# Autodesk Inventor assembly: Wolley Wheel
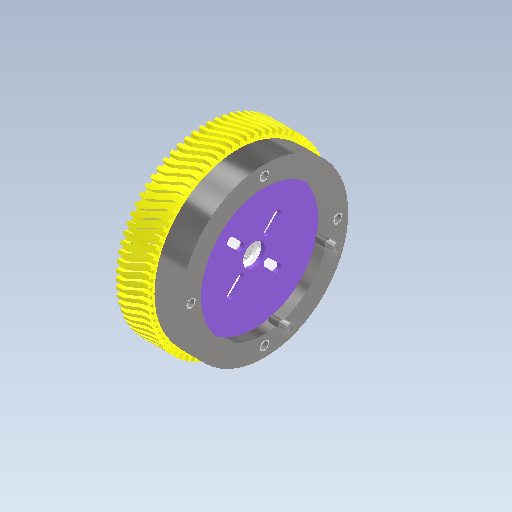
[picture p0: Inventor's stored thumbnail of the model, 512x512]
Saved by Autodesk Inventor 2021 (Build 250183000, 183)
## iProperties
Created: 2021-02-27
Part Number: Wolley Wheel
Document SubType Name: Assembly
Designer: Jack
Author: Jack
Title: Wolley Wheel
## Documents named in this file (37)
- C:\Users\Jack\Projekt\Wolley\MEC_SpeedReducerWheel\SpeedReducerWheel.iam
- C:\Users\Jack\Projekt\Wolley\MEC_SpeedReducerWheel\Back.ipt
- C:\Users\Jack\Projekt\Wolley\MEC_SpeedReducerWheel\RingGearA.ipt
- C:\Users\Jack\Projekt\Wolley\MEC_SpeedReducerWheel\SunGearA.ipt
- C:\Users\Jack\Projekt\Wolley\MEC_SpeedReducerWheel\PlanetGearA.ipt
- C:\Users\Jack\Projekt\Wolley\MEC_SpeedReducerWheel\Middle.ipt
- C:\Users\Jack\Projekt\Wolley\MEC_SpeedReducerWheel\PCB.ipt
- C:\Users\Jack\Projekt\Wolley\MEC_SpeedReducerWheel\Carrier.ipt
- C:\Users\Jack\Projekt\Wolley\MEC_SpeedReducerWheel\Shaft1.ipt
- C:\Users\Jack\Projekt\Wolley\MEC_SpeedReducerWheel\Shaft2.ipt
- C:\Users\Jack\Projekt\Wolley\MEC_SpeedReducerWheel\CarrierB.ipt
- C:\Users\Jack\Projekt\Wolley\MEC_SpeedReducerWheel\Front.ipt
- C:\Users\Jack\Projekt\Wolley\MEC_SpeedReducerWheel\Wheel.ipt
- C:\Users\Jack\Projekt\Wolley\MEC_SpeedReducerWheel\SunGearB.ipt
- C:\Users\Jack\Projekt\Wolley\MEC_SpeedReducerWheel\Tire.ipt
- C:\Users\Jack\Projekt\Wolley\MEC_SpeedReducerWheel\Enclosure.ipt
- C:\Users\Jack\Projekt\Wolley\MEC_SpeedReducerWheel\PlanetGearB.ipt
- C:\Users\Jack\Projekt\Wolley\MEC_SpeedReducerWheel\Mount.ipt
- C:\Users\Jack\Projekt\Wolley\MEC_SpeedReducerWheel\SpeedReducerWheel\Design Accelerator\RingGearA_SpurGears.iam
- C:\Users\Jack\Projekt\Wolley\MEC_SpeedReducerWheel\SpeedReducerWheel\Design Accelerator\PlanetGearA_SpurGears2.iam
- C:\Users\Jack\Projekt\Wolley\MEC_SpeedReducerWheel\SpeedReducerWheel\Design Accelerator\SunGearB_SpurGears1.iam
- C:\Users\Jack\Projekt\Wolley\MEC_SpeedReducerWheel\SpeedReducerWheel\Design Accelerator\PlanetGearB_SpurGears1.iam
- C:\Users\Jack\Projekt\Wolley\MEC_SpeedReducerWheel\SpeedReducerWheel\Design Accelerator\RingGearB_SpurGears.iam
- C:\Users\Jack\Projekt\Wolley\MEC_SpeedReducerWheel\PlanetGearB_CPY.ipt
- C:\Users\Jack\Projekt\Wolley\MEC_SpeedReducerWheel\PlanetGearB_CPY1.ipt
- C:\Users\Jack\Documents\Inventor\Content Center Files\R2021\en-US\DIN 912\DIN 912 - M3 x 0,5 x 5 x 3,75.ipt
- C:\Users\Jack\Projekt\Wolley\MEC_SpeedReducerWheel\MiddleStandoff.ipt
- C:\Users\Jack\Projekt\Wolley\MEC_SpeedReducerWheel\SpeedReducerWheel\Design Accelerator\SunGearA_SpurGears2.iam
- C:\Users\Jack\Projekt\Wolley\MEC_SpeedReducerWheel\Shaft1_1.ipt
- C:\Users\Jack\Projekt\Wolley\MEC_SpeedReducerWheel\Magnet.ipt
- C:\Users\Jack\Projekt\Wolley\MEC_SpeedReducerWheel\Magnet_CPY.ipt
- C:\Users\Jack\Projekt\Wolley\MEC_SpeedReducerWheel\Magnet_CPY1.ipt
- C:\Users\Jack\Documents\Inventor\Content Center Files\R2021\en-US\DIN 912\DIN 912 - M3 x 0,5 x 6 x 4,75.ipt
- C:\Users\Jack\Projekt\Wolley\MEC_SpeedReducerWheel\PlanetGearA_CPY2.ipt
- C:\Users\Jack\Projekt\Wolley\MEC_SpeedReducerWheel\PlanetGearA_CPY3.ipt
- C:\Users\Jack\Documents\Inventor\Content Center Files\R2021\en-US\DIN 912\DIN 912 - M3 x 0,5 x 16 x 14,75.ipt
- C:\Users\Jack\Projekt\Wolley\MEC_SpeedReducerWheel\M3ThreadedInsert.ipt
## Components (54 placed, 36 different names)
1. Back:1
2. RingGearA:1
3. SunGearA:1 — Flush:1, Mate:2
4. PlanetGearA:1 — Rotational:1, Flush:1
5. Middle:1 — Mate:1, Rotational:5, Rotational:6, Insert:1, Insert:2, Insert:3, Rotational:16, Rotational:17, Rotational:18, Insert:4, Insert:5, Insert:6, Insert:7
6. PCB:1
7. Carrier:1 — Rotational:1, Rigid:2, Rigid:3, Rigid:4, Rotational:19, Rotational:20
8. Shaft1:1
9. Shaft2:1
10. CarrierB:1 — Mate:3, Mate:5, Mate:7, Rotational:9, Rotational:10, Rotational:11
11. Front:1 — Mate:4, Mate:6, Mate:8
12. Wheel:1 — Rotational:6, Rigid:1
13. SunGearB:1 — Rotational:5
14. Tire:1 — Rigid:1
15. Enclosure:1 — Rigid:5, Rigid:6, Rigid:7, Rigid:8
16. PlanetGearB:1 — Rotational:9
17. Mount:1
18. RingGearA_SpurGears:1 [sub-assembly]
19. PlanetGearA_SpurGears:1 [sub-assembly]
20. SunGearB_SpurGears:1 [sub-assembly]
21. PlanetGearB_SpurGears:1 [sub-assembly]
22. RingGearB_SpurGears:1 [sub-assembly]
23. PlanetGearB_CPY:1 — Rotational:10
24. PlanetGearB_CPY1:1 — Rotational:11
25. DIN 912 - replaced by DIN EN ISO 4762 M3 x 5:1 — Mate:3, Mate:4
26. DIN 912 - replaced by DIN EN ISO 4762 M3 x 5:2 — Mate:5, Mate:6
27. DIN 912 - replaced by DIN EN ISO 4762 M3 x 5:3 — Mate:7, Mate:8
28. DIN 912 - replaced by DIN EN ISO 4762 M3 x 5:4 — Insert:1
29. DIN 912 - replaced by DIN EN ISO 4762 M3 x 5:5 — Insert:2
30. DIN 912 - replaced by DIN EN ISO 4762 M3 x 5:6 — Insert:3
31. SunGearA_SpurGears2:1 [sub-assembly]
32. Shaft1_1:1
33. Magnet:1 — Rigid:2
34. Magnet_CPY:1 — Rigid:3
35. Magnet_CPY1:1 — Rigid:4
36. DIN 912 - replaced by DIN EN ISO 4762 M3 x 6:3
37. DIN 912 - replaced by DIN EN ISO 4762 M3 x 6:4
38. MiddleStandoff:9 — Rotational:16
39. MiddleStandoff:10 — Rotational:17
40. MiddleStandoff:11 — Rotational:18
41. PlanetGearA_CPY2:1 — Rotational:19
42. PlanetGearA_CPY3:1 — Rotational:20
43. DIN 912 - replaced by DIN EN ISO 4762 M3 x 16:1 — Insert:4
44. DIN 912 - replaced by DIN EN ISO 4762 M3 x 16:2 — Insert:5
45. DIN 912 - replaced by DIN EN ISO 4762 M3 x 16:3 — Insert:6
46. DIN 912 - replaced by DIN EN ISO 4762 M3 x 16:4 — Insert:7
47. M3ThreadedInsert:1 — Rigid:5
48. M3ThreadedInsert:2 — Rigid:6
49. M3ThreadedInsert:3 — Rigid:7
50. M3ThreadedInsert:4 — Rigid:8
51. MiddleStandoff:1
52. MiddleStandoff:2
53. MiddleStandoff:3
54. MiddleStandoff:4
## Component patterns: (4 elements, first: MiddleStandoff:1)
## Relationships (35: RevoluteJoint 11, Mate 8, WeldJoint 8, Insert 7, Flush 1)
- Rotational:1 [RevoluteJoint] (1 mm): PlanetGearA:1 ↔ Carrier:1
- Mate:1: Middle:1
- Flush:1: SunGearA:1 ↔ PlanetGearA:1
- Mate:2: SunGearA:1
- Rotational:5 [RevoluteJoint]: Middle:1 ↔ SunGearB:1
- Rotational:6 [RevoluteJoint]: Middle:1 ↔ Wheel:1
- Rigid:1 [WeldJoint]: Wheel:1 ↔ Tire:1
- Mate:3: CarrierB:1 ↔ DIN 912 - replaced by DIN EN ISO 4762 M3 x 5:1
- Mate:4: Front:1 ↔ DIN 912 - replaced by DIN EN ISO 4762 M3 x 5:1
- Mate:5: CarrierB:1 ↔ DIN 912 - replaced by DIN EN ISO 4762 M3 x 5:2
- Mate:6: Front:1 ↔ DIN 912 - replaced by DIN EN ISO 4762 M3 x 5:2
- Mate:7: CarrierB:1 ↔ DIN 912 - replaced by DIN EN ISO 4762 M3 x 5:3
- Mate:8: Front:1 ↔ DIN 912 - replaced by DIN EN ISO 4762 M3 x 5:3
- Insert:1: Middle:1 ↔ DIN 912 - replaced by DIN EN ISO 4762 M3 x 5:4
- Insert:2: Middle:1 ↔ DIN 912 - replaced by DIN EN ISO 4762 M3 x 5:5
- Insert:3: Middle:1 ↔ DIN 912 - replaced by DIN EN ISO 4762 M3 x 5:6
- Rotational:9 [RevoluteJoint]: CarrierB:1 ↔ PlanetGearB:1
- Rotational:10 [RevoluteJoint]: CarrierB:1 ↔ PlanetGearB_CPY:1
- Rotational:11 [RevoluteJoint]: CarrierB:1 ↔ PlanetGearB_CPY1:1
- Rigid:2 [WeldJoint]: Carrier:1 ↔ Magnet:1
- Rigid:3 [WeldJoint]: Carrier:1 ↔ Magnet_CPY:1
- Rigid:4 [WeldJoint]: Carrier:1 ↔ Magnet_CPY1:1
- Rotational:16 [RevoluteJoint]: Middle:1 ↔ MiddleStandoff:9
- Rotational:17 [RevoluteJoint]: Middle:1 ↔ MiddleStandoff:10
- Rotational:18 [RevoluteJoint]: Middle:1 ↔ MiddleStandoff:11
- Rotational:19 [RevoluteJoint]: Carrier:1 ↔ PlanetGearA_CPY2:1
- Rotational:20 [RevoluteJoint]: Carrier:1 ↔ PlanetGearA_CPY3:1
- Insert:4: Middle:1 ↔ DIN 912 - replaced by DIN EN ISO 4762 M3 x 16:1
- Insert:5: Middle:1 ↔ DIN 912 - replaced by DIN EN ISO 4762 M3 x 16:2
- Insert:6: Middle:1 ↔ DIN 912 - replaced by DIN EN ISO 4762 M3 x 16:3
- Insert:7: Middle:1 ↔ DIN 912 - replaced by DIN EN ISO 4762 M3 x 16:4
- Rigid:5 [WeldJoint]: Enclosure:1 ↔ M3ThreadedInsert:1
- Rigid:6 [WeldJoint]: Enclosure:1 ↔ M3ThreadedInsert:2
- Rigid:7 [WeldJoint]: Enclosure:1 ↔ M3ThreadedInsert:3
- Rigid:8 [WeldJoint]: Enclosure:1 ↔ M3ThreadedInsert:4
